# Autodesk Inventor assembly: Ankle
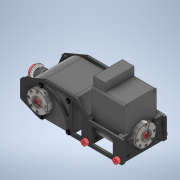
[picture p0: Inventor's stored thumbnail of the model, 180x180]
Saved by Autodesk Inventor 2022.3 (Build 263350000, 350)
## iProperties
Created: 2023-05-14
Part Number: Ankle
Document SubType Name: Assembly
Designer: Masato Kubotera
Mass: 250.631 g
Surface Area: 693.673 cm^2
Volume: 230.731 cm^3
Density: 1.08625 g/cm^3
Author: Masato Kubotera
## Documents named in this file (16)
- C:\Users\Masato\Documents\Inventor\Inventor for CIT Brains\SUSTAINA-OP - ankle\LowerBody\Ankle\Ankle.iam
- C:\Users\Masato\Documents\Inventor\Inventor for CIT Brains\SUSTAINA-OP - ankle\LowerBody\Ankle\Ankle_side_frame.ipt
- C:\Users\Masato\Documents\Inventor\Inventor for CIT Brains\SUSTAINA-OP - ankle\ReadyMade\KONDO\B3M-SC-1170-A_with_ClampHorn_AND_FreeHorn.iam
- C:\Users\Masato\Documents\Inventor\Inventor for CIT Brains\SUSTAINA-OP - ankle\ReadyMade\KONDO\B3M-SC-1040-A_with_ClampHorn.iam
- C:\Users\Masato\Documents\Inventor\Inventor for CIT Brains\SUSTAINA-OP - ankle\LowerBody\Ankle\Ankle_back_frame.ipt
- C:\Users\Masato\Documents\Inventor\Inventor for CIT Brains\SUSTAINA-OP - ankle\ReadyMade\Screw\F-2615EB.ipt
- C:\Users\Masato\Documents\Inventor\Inventor for CIT Brains\SUSTAINA-OP - ankle\ReadyMade\Screw\F-2620EB.ipt
- C:\Users\Masato\Documents\Inventor\Inventor for CIT Brains\SUSTAINA-OP - ankle\ReadyMade\Screw\UC-0306.ipt
- C:\Users\Masato\Documents\Inventor\Inventor for CIT Brains\SUSTAINA-OP - ankle\ReadyMade\Screw\FC-2615EB.ipt
- C:\Users\Masato\Documents\Inventor\Inventor for CIT Brains\SUSTAINA-OP - ankle\LowerBody\Ankle\Ankle_front_frame.iam
- C:\Users\Masato\Documents\Inventor\Inventor for CIT Brains\SUSTAINA-OP - ankle\ReadyMade\Washer\UUW-0412-20H.ipt
- C:\Users\Masato\Documents\Inventor\Inventor for CIT Brains\SUSTAINA-OP - ankle\ReadyMade\Washer\CC-0612-15B.ipt
- C:\Users\Masato\Documents\Inventor\Inventor for CIT Brains\SUSTAINA-OP - ankle\ReadyMade\Bush\80F-0603.ipt
- C:\Users\Masato\Documents\Inventor\Inventor for CIT Brains\SUSTAINA-OP - ankle\ReadyMade\Screw\DBTS4-7-5-DHC.ipt
- C:\Users\Masato\Documents\Inventor\Inventor for CIT Brains\SUSTAINA-OP - ankle\ReadyMade\Washer\UUW-0614-03H.ipt
- C:\Users\Masato\Documents\Inventor\Inventor for CIT Brains\SUSTAINA-OP - ankle\ReadyMade\Washer\TT-0814-10.ipt
## Components (27 placed, 15 different names)
1. Ankle_front_frame:1 [sub-assembly] — メイト:1, メイト:2, メイト:3, 挿入:29
2. Ankle_side_frame:1 — 挿入:1, 挿入:2, 挿入:3, 挿入:4, 挿入:9, 挿入:11, 挿入:15, 挿入:16, 挿入:17, 挿入:18, 挿入:23, 挿入:25, メイト:1, メイト:2, メイト:3
3. Ankle_side_frame:2 — 挿入:5, 挿入:6, 挿入:7, 挿入:8, 挿入:10, 挿入:12, 挿入:19, 挿入:20, 挿入:21, 挿入:22, 挿入:24, 挿入:26
4. Ankle_back_frame:1 — 挿入:11, 挿入:12, 角度:1, 挿入:13, 挿入:14, 挿入:27, 挿入:28
5. Ankle_back_frame:2 — 挿入:9, 挿入:10, 角度:2
6. UUW-0412-20H:1 — 挿入:29, 挿入:30, 挿入:32
7. CC-0612-15B:1 — 挿入:30, 挿入:31
8. 80F-0603:1 — 挿入:31
9. DBTS4-7-5-DHC:1 — 挿入:32, 挿入:33
10. UUW-0614-03H:1 — 挿入:33, 挿入:34
11. TT-0814-10:1 — 挿入:34
12. B3M-SC-1170-A_with_ClampHorn_AND_FreeHorn:1 [sub-assembly] — 挿入:1, 挿入:2, 挿入:3, 挿入:4, 挿入:5, 挿入:6, 挿入:7, 挿入:8, メイト:4
13. B3M-SC-1040-A_with_ClampHorn:1 [sub-assembly] — 挿入:13, 挿入:14, フラッシュ:1, フラッシュ:2
14. F-2615EB:1 — 挿入:15
15. F-2615EB:2 — 挿入:16
16. F-2615EB:3 — 挿入:17
17. F-2615EB:4 — 挿入:18
18. F-2620EB:1 — 挿入:19
19. F-2620EB:2 — 挿入:20
20. F-2620EB:3 — 挿入:21
21. F-2620EB:4 — 挿入:22
22. UC-0306:1 — 挿入:23
23. UC-0306:2 — 挿入:24
24. UC-0306:3 — 挿入:25
25. UC-0306:4 — 挿入:26
26. FC-2615EB:1 — 挿入:27
27. FC-2615EB:2 — 挿入:28
## Relationships (42: Insert 34, Mate 4, Angle 2, Flush 2)
- 挿入:1 [Insert]: Ankle_side_frame:1 ↔ B3M-SC-1170-A_with_ClampHorn_AND_FreeHorn:1
- 挿入:2 [Insert]: Ankle_side_frame:1 ↔ B3M-SC-1170-A_with_ClampHorn_AND_FreeHorn:1
- 挿入:3 [Insert]: Ankle_side_frame:1 ↔ B3M-SC-1170-A_with_ClampHorn_AND_FreeHorn:1
- 挿入:4 [Insert]: Ankle_side_frame:1 ↔ B3M-SC-1170-A_with_ClampHorn_AND_FreeHorn:1
- 挿入:5 [Insert]: Ankle_side_frame:2 ↔ B3M-SC-1170-A_with_ClampHorn_AND_FreeHorn:1
- 挿入:6 [Insert]: Ankle_side_frame:2 ↔ B3M-SC-1170-A_with_ClampHorn_AND_FreeHorn:1
- 挿入:7 [Insert]: Ankle_side_frame:2 ↔ B3M-SC-1170-A_with_ClampHorn_AND_FreeHorn:1
- 挿入:8 [Insert]: Ankle_side_frame:2 ↔ B3M-SC-1170-A_with_ClampHorn_AND_FreeHorn:1
- 挿入:9 [Insert]: Ankle_side_frame:1 ↔ Ankle_back_frame:2
- 挿入:10 [Insert]: Ankle_side_frame:2 ↔ Ankle_back_frame:2
- 挿入:11 [Insert]: Ankle_side_frame:1 ↔ Ankle_back_frame:1
- 挿入:12 [Insert]: Ankle_side_frame:2 ↔ Ankle_back_frame:1
- 角度:1 [Angle] (0 deg): Ankle_back_frame:1
- 角度:2 [Angle] (0 deg): Ankle_back_frame:2
- 挿入:13 [Insert]: Ankle_back_frame:1 ↔ B3M-SC-1040-A_with_ClampHorn:1
- 挿入:14 [Insert]: Ankle_back_frame:1 ↔ B3M-SC-1040-A_with_ClampHorn:1
- 挿入:15 [Insert]: Ankle_side_frame:1 ↔ F-2615EB:1
- 挿入:16 [Insert]: Ankle_side_frame:1 ↔ F-2615EB:2
- 挿入:17 [Insert]: Ankle_side_frame:1 ↔ F-2615EB:3
- 挿入:18 [Insert]: Ankle_side_frame:1 ↔ F-2615EB:4
- 挿入:19 [Insert]: Ankle_side_frame:2 ↔ F-2620EB:1
- 挿入:20 [Insert]: Ankle_side_frame:2 ↔ F-2620EB:2
- 挿入:21 [Insert]: Ankle_side_frame:2 ↔ F-2620EB:3
- 挿入:22 [Insert]: Ankle_side_frame:2 ↔ F-2620EB:4
- 挿入:23 [Insert]: Ankle_side_frame:1 ↔ UC-0306:1
- 挿入:24 [Insert]: Ankle_side_frame:2 ↔ UC-0306:2
- 挿入:25 [Insert]: Ankle_side_frame:1 ↔ UC-0306:3
- 挿入:26 [Insert]: Ankle_side_frame:2 ↔ UC-0306:4
- 挿入:27 [Insert]: Ankle_back_frame:1 ↔ FC-2615EB:1
- 挿入:28 [Insert]: Ankle_back_frame:1 ↔ FC-2615EB:2
- メイト:1 [Mate] (0.025 mm): Ankle_front_frame:1 ↔ Ankle_side_frame:1
- メイト:2 [Mate] (0.025 mm): Ankle_front_frame:1 ↔ Ankle_side_frame:1
- メイト:3 [Mate]: Ankle_front_frame:1 ↔ Ankle_side_frame:1
- 挿入:29 [Insert]: Ankle_front_frame:1 ↔ UUW-0412-20H:1
- 挿入:30 [Insert]: UUW-0412-20H:1 ↔ CC-0612-15B:1
- 挿入:31 [Insert]: CC-0612-15B:1 ↔ 80F-0603:1
- 挿入:32 [Insert]: UUW-0412-20H:1 ↔ DBTS4-7-5-DHC:1
- 挿入:33 [Insert]: DBTS4-7-5-DHC:1 ↔ UUW-0614-03H:1
- 挿入:34 [Insert]: UUW-0614-03H:1 ↔ TT-0814-10:1
- メイト:4 [Mate]: B3M-SC-1170-A_with_ClampHorn_AND_FreeHorn:1
- フラッシュ:1 [Flush]: B3M-SC-1040-A_with_ClampHorn:1
- フラッシュ:2 [Flush]: B3M-SC-1040-A_with_ClampHorn:1
